# Autodesk Inventor assembly: Road Grip Thick and not assembled
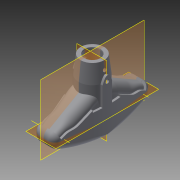
[picture p0: Inventor's stored thumbnail of the model, 180x180]
Saved by Autodesk Inventor 2018.2 (Build 222227000, 227)
## iProperties
Created: 2018-02-16
Part Number: Road Grip Thick and not assembled
Document SubType Name: Assembly
Designer: Rus
Author: Rus
## Documents named in this file (3)
- E:\Libraries\3D Objects\Longboard\Land Paddle\Road Grip\V0.0\Road Grip Thick and not assembled.iam
- E:\Libraries\3D Objects\Longboard\Land Paddle\Road Grip\V0.0\Road Grip.ipt
- E:\Libraries\3D Objects\Longboard\Land Paddle\Road Grip\V0.0\Road Grip Thick.ipt
## Components (2 placed, 2 different names)
1. Road Grip:1 — Insert:1, Flush:1
2. Road Grip Thick:1 — Insert:1, Flush:1
## Relationships (2: Insert 1, Flush 1)
- Insert:1: Road Grip:1 ↔ Road Grip Thick:1
- Flush:1: Road Grip:1 ↔ Road Grip Thick:1
